# Autodesk Inventor assembly: ROUNDCIRCUITBOARD
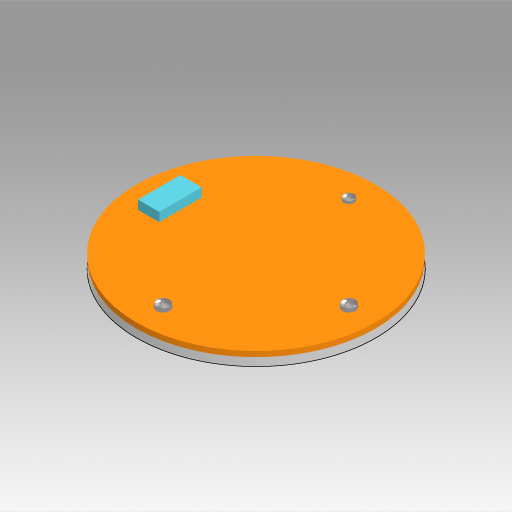
[picture p0: Inventor's stored thumbnail of the model, 512x512]
Saved by Autodesk Inventor 2023 (Build 270158000, 158)
## iProperties
Created: 2025-09-17
Part Number: ROUNDCIRCUITBOARD
Document SubType Name: Assembly
Designer: NELLY NDUNG'U
Author: NELLY NDUNG'U
## Documents named in this file (6)
- N:\NNW\PLC_PROJECTS\SPOTLIGHT PROJECT\ROUNDCIRCUITBOARD.iam
- N:\NNW\PLC_PROJECTS\SPOTLIGHT PROJECT\ROUNDBOTTOMCOVER.ipt
- N:\NNW\PLC_PROJECTS\SPOTLIGHT PROJECT\ROUNDPCB.ipt
- N:\NNW\PLC_PROJECTS\SPOTLIGHT PROJECT\ROUNDTOPCOVER.ipt
- C:\Users\User\OneDrive\Documents\Inventor\Content Center Files\R2023\en-US\ANSI B18.6.5M(24)\ANSI B18.6.5M - M2.5x0.45 x 4(36).ipt
- C:\Users\User\OneDrive\Documents\Inventor\Content Center Files\R2023\en-US\ANSI B18.6.5M(24)\ANSI B18.6.5M - M2x0.4 x 4(36).ipt
## Components (6 placed, 5 different names)
1. ROUNDBOTTOMCOVER:1 — Insert:1, Mate:1
2. ROUNDPCB:1 — Insert:1
3. ROUNDTOPCOVER:1 — Mate:1, Insert:2, Insert:3, Insert:4
4. Cross Recessed Pan Head Tapping Screw - Type F - Type I - Metric M2x0.4 x 4:1 — Insert:2
5. Cross Recessed Pan Head Tapping Screw - Type F - Type I - Metric M2.5x0.45 x 4:2 — Insert:3
6. Cross Recessed Pan Head Tapping Screw - Type F - Type I - Metric M2.5x0.45 x 4:3 — Insert:4
## Relationships (5: Insert 4, Mate 1)
- Insert:1: ROUNDBOTTOMCOVER:1 ↔ ROUNDPCB:1
- Mate:1: ROUNDBOTTOMCOVER:1 ↔ ROUNDTOPCOVER:1
- Insert:2: ROUNDTOPCOVER:1 ↔ Cross Recessed Pan Head Tapping Screw - Type F - Type I - Metric M2x0.4 x 4:1
- Insert:3: ROUNDTOPCOVER:1 ↔ Cross Recessed Pan Head Tapping Screw - Type F - Type I - Metric M2.5x0.45 x 4:2
- Insert:4: ROUNDTOPCOVER:1 ↔ Cross Recessed Pan Head Tapping Screw - Type F - Type I - Metric M2.5x0.45 x 4:3
